# Autodesk Inventor assembly: 21700_5s_1p
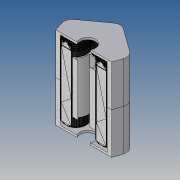
[picture p0: Inventor's stored thumbnail of the model, 180x180]
Saved by Autodesk Inventor 2019.4 (Build 234330000, 330)
## iProperties
Part Number: 21700_5s_1p
Document SubType Name: Assembly
Designer: Admin
Mass: 421.089 g
Surface Area: 465.946 cm^2
Volume: 53.5737 cm^3
Density: 7.86 g/cm^3
Author: Admin
Revision: -
VAULT_Status: in Bearbeitung
Gewicht: 0,421 kg
InventorVersion: 2019.4
Volumen: 53573,698
## Documents named in this file (5)
- C:\Users\tonn\Documents\GitHub\CAD_Elements\Hilfsdateien\21700_5s_1p.iam
- Norm.iam
- C:\Users\tonn\Documents\GitHub\CAD_Elements\CAD\Hektor\Hektor_3D\21700_li_battery.ipt
- C:\Users\tonn\Documents\GitHub\CAD_Elements\CAD\Zubehör\21700_stern.ipt
- C:\Users\tonn\Documents\GitHub\CAD_Elements\CAD\Zubehör\21700_case.ipt
## Components (8 placed, 3 different names)
1. 21700_stern:1 — Passend:1, Passend:2, Passend:3, Passend:4, Passend:5, Fluchtend:5, Passend:6, Passend:7
2. 21700_li_battery:1 — Passend:3, Fluchtend:3
3. 21700_li_battery:2 — Passend:2, Fluchtend:1, Fluchtend:5, Passend:9
4. 21700_li_battery:3 — Passend:4, Fluchtend:1, Fluchtend:2, Fluchtend:3, Fluchtend:4
5. 21700_li_battery:4 — Passend:5, Fluchtend:2
6. 21700_li_battery:5 — Passend:1, Fluchtend:4
7. 21700_case:1 — Passend:8, Passend:9, Winkel:1, Fluchtend:6, Passend:11
8. 21700_case:2 — Fluchtend:6, Passend:10, Passend:11
## Relationships (18: Mate 11, Flush 6, Angle 1)
- Passend:1 [Mate]: 21700_stern:1 ↔ 21700_li_battery:5
- Passend:2 [Mate]: 21700_stern:1 ↔ 21700_li_battery:2
- Passend:3 [Mate]: 21700_stern:1 ↔ 21700_li_battery:1
- Passend:4 [Mate]: 21700_stern:1 ↔ 21700_li_battery:3
- Passend:5 [Mate]: 21700_stern:1 ↔ 21700_li_battery:4
- Fluchtend:1 [Flush]: 21700_li_battery:2 ↔ 21700_li_battery:3
- Fluchtend:2 [Flush]: 21700_li_battery:3 ↔ 21700_li_battery:4
- Fluchtend:3 [Flush]: 21700_li_battery:1 ↔ 21700_li_battery:3
- Fluchtend:4 [Flush]: 21700_li_battery:3 ↔ 21700_li_battery:5
- Fluchtend:5 [Flush] (-10 mm): 21700_stern:1 ↔ 21700_li_battery:2
- Passend:6 [Mate]: 21700_stern:1
- Passend:7 [Mate]: 21700_stern:1
- Passend:8 [Mate]: 21700_case:1
- Passend:9 [Mate] (3 mm): 21700_li_battery:2 ↔ 21700_case:1
- Winkel:1 [Angle] (0 deg): 21700_case:1
- Fluchtend:6 [Flush]: 21700_case:1 ↔ 21700_case:2
- Passend:10 [Mate]: 21700_case:2
- Passend:11 [Mate]: 21700_case:1 ↔ 21700_case:2
## Named parameters: Gewicht = 0.421089, Volumen = 53.5737
note: some values were not read from the file. Shown as the stored number, unit unknown: "Gewicht", "Volumen".
